# Autodesk Inventor assembly: ApertureActuator
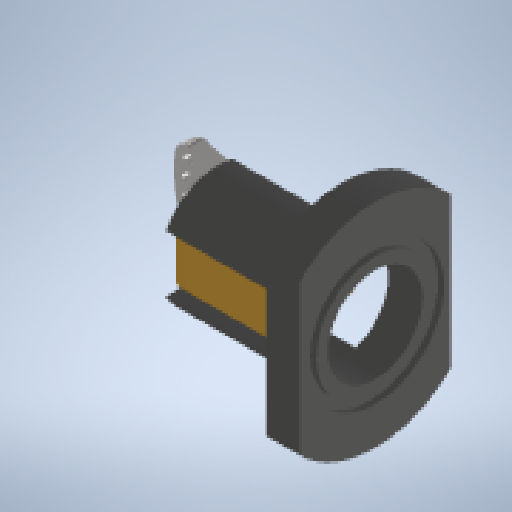
[picture p0: Inventor's stored thumbnail of the model, 512x512]
Saved by Autodesk Inventor 2023 (Build 270158000, 158)
## iProperties
Created: 2022-04-02
Part Number: ApertureActuator
Document SubType Name: Assembly
Designer: Vinicius Miguel
Author: Vinicius Miguel
## Documents named in this file (4)
- P:\SEM-Mechanical\ApertureActuator.iam
- P:\SEM-Mechanical\022.ipt
- P:\SEM-Mechanical\023.ipt
- P:\SEM-Mechanical\GM1024BY10.ipt
## Components (3 placed, 3 different names)
1. 022:1 — Flush:1, Mate:3, Flush:2, Angle:1
2. 023:1 — Mate:4, Flush:3, Angle:1
3. GM1024BY10:1 — Flush:1, Mate:3, Flush:2, Mate:4, Flush:3
## Relationships (6: Flush 3, Mate 2, Angle 1)
- Flush:1: 022:1 ↔ GM1024BY10:1
- Mate:3: 022:1 ↔ GM1024BY10:1
- Flush:2: 022:1 ↔ GM1024BY10:1
- Mate:4: 023:1 ↔ GM1024BY10:1
- Flush:3: 023:1 ↔ GM1024BY10:1
- Angle:1 (5 deg): 022:1 ↔ 023:1
